# Autodesk Inventor assembly: pms7003
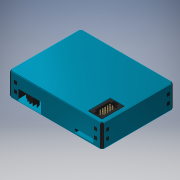
[picture p0: Inventor's stored thumbnail of the model, 180x180]
Saved by Autodesk Inventor 2018 (Build 220112000, 112)
## iProperties
Created: 2017-08-15
Part Number: pms7003
Document SubType Name: Assembly
Designer: ZEUSLAP
Sending System: SolidWorks 2017
Last Author: Adrian
Last Saved: 2017-08-15
Author: ZEUSLAP
## Documents named in this file (7)
- C:\Users\ZEUSLAP\YandexDisk\Inventor\comparative_air_pollution_sensor\module_pms7003\parts\plantower-pms7003-laser-dust-sensor\pms7003.iam
- C:\Users\ZEUSLAP\YandexDisk\Inventor\comparative_air_pollution_sensor\module_pms7003\parts\plantower-pms7003-laser-dust-sensor\parts\fan.ipt
- C:\Users\ZEUSLAP\YandexDisk\Inventor\comparative_air_pollution_sensor\module_pms7003\parts\plantower-pms7003-laser-dust-sensor\parts\plastic.ipt
- C:\Users\ZEUSLAP\YandexDisk\Inventor\comparative_air_pollution_sensor\module_pms7003\parts\plantower-pms7003-laser-dust-sensor\parts\metal_cover_connector.ipt
- C:\Users\ZEUSLAP\YandexDisk\Inventor\comparative_air_pollution_sensor\module_pms7003\parts\plantower-pms7003-laser-dust-sensor\parts\metal_cover_fan.ipt
- C:\Users\ZEUSLAP\YandexDisk\Inventor\comparative_air_pollution_sensor\module_pms7003\parts\plantower-pms7003-laser-dust-sensor\parts\1_27mm_Header\1_27mm_2x10pin.iam
- 1_27mm_2x5pin.iam
## Components (5 placed, 5 different names)
1. fan:1 — Angle:1, Mate:1, Mate:2, Mate:3
2. plastic:1 — Angle:1, Mate:1, Mate:2, Mate:3, Mate:4, Mate:5, Mate:7, Mate:8, Mate:10, Flush:2, Mate:12, Mate:13
3. metal_cover_connector:1 — Mate:4, Mate:5, Mate:6, Angle:2, Mate:7, Mate:9
4. metal_cover_fan:1 — Mate:8, Mate:9, Mate:10, Mate:11, Flush:1
5. 1_27mm_2x5pin:1 [sub-assembly] — Angle:3, Flush:2, Mate:12, Mate:13
## Relationships (18: Mate 13, Angle 3, Flush 2)
- Angle:1 (180 deg): fan:1 ↔ plastic:1
- Mate:1: fan:1 ↔ plastic:1
- Mate:2 (7.5 mm): fan:1 ↔ plastic:1
- Mate:3 (7.5 mm): fan:1 ↔ plastic:1
- Mate:4: plastic:1 ↔ metal_cover_connector:1
- Mate:5: plastic:1 ↔ metal_cover_connector:1
- Mate:6: metal_cover_connector:1
- Angle:2 (180 deg): metal_cover_connector:1
- Mate:7: plastic:1 ↔ metal_cover_connector:1
- Mate:8: plastic:1 ↔ metal_cover_fan:1
- Mate:9: metal_cover_connector:1 ↔ metal_cover_fan:1
- Mate:10: plastic:1 ↔ metal_cover_fan:1
- Mate:11: metal_cover_fan:1
- Flush:1 (22 mm): metal_cover_fan:1
- Angle:3 (270 deg): 1_27mm_2x5pin:1
- Flush:2 (0.3 mm): plastic:1 ↔ 1_27mm_2x5pin:1
- Mate:12 (1.4 mm): plastic:1 ↔ 1_27mm_2x5pin:1
- Mate:13 (2.6 mm): plastic:1 ↔ 1_27mm_2x5pin:1
